# Autodesk Inventor assembly: FULL
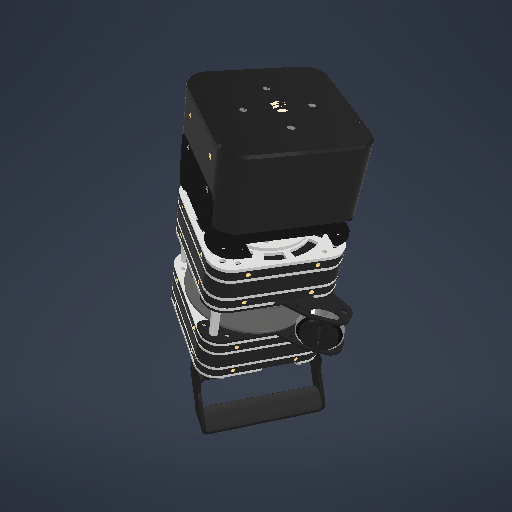
[picture p0: Inventor's stored thumbnail of the model, 512x512]
Saved by Autodesk Inventor 2026.1 (Build 301233000, 233)
## iProperties
Created: 2025-03-02
Part Number: FULL
Document SubType Name: Assembly
Designer: aaron
Author: aaron
## Documents named in this file (5)
- D:\work\loopandpixel\openworkoutsystem\cad\v5\FULL.iam
- D:\work\loopandpixel\openworkoutsystem\cad\v5\drivetrain.iam
- D:\work\loopandpixel\openworkoutsystem\cad\v5\battery_pack_16s.ipt.iam
- C:\Users\aaron\OneDrive\Documents\Inventor\Content Center Files\R2026\en-US\IS 6761\IS 6761 - M3 x 8 - 0.5.ipt
- battery_pack_16s.ipt
## Components (8 placed, 3 different names)
1. battery_pack_16s.ipt:1 [sub-assembly] — Flush:1, Flush:2, Mate:1
2. drivetrain:2 [sub-assembly] — Flush:1, Flush:2, Mate:1, Mate:2, Mate:3, Mate:4, Mate:5, Mate:6, Mate:7
3. IS 6761 M3 x 8:1 — Mate:2
4. IS 6761 M3 x 8:2 — Mate:3
5. IS 6761 M3 x 8:3 — Mate:4
6. IS 6761 M3 x 8:4 — Mate:5
7. IS 6761 M3 x 8:5 — Mate:6
8. IS 6761 M3 x 8:6 — Mate:7
## Relationships (9: Mate 7, Flush 2)
- Flush:1: battery_pack_16s.ipt:1 ↔ drivetrain:2
- Flush:2: battery_pack_16s.ipt:1 ↔ drivetrain:2
- Mate:1: battery_pack_16s.ipt:1 ↔ drivetrain:2
- Mate:2: drivetrain:2 ↔ IS 6761 M3 x 8:1
- Mate:3: drivetrain:2 ↔ IS 6761 M3 x 8:2
- Mate:4: drivetrain:2 ↔ IS 6761 M3 x 8:3
- Mate:5: drivetrain:2 ↔ IS 6761 M3 x 8:4
- Mate:6: drivetrain:2 ↔ IS 6761 M3 x 8:5
- Mate:7: drivetrain:2 ↔ IS 6761 M3 x 8:6
